# Autodesk Inventor assembly: motor_sima
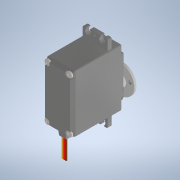
[picture p0: Inventor's stored thumbnail of the model, 180x180]
Saved by Autodesk Inventor 2020.3 (Build 243373000, 373)
## iProperties
Created: 2019-08-01
Part Number: motor_sima
Document SubType Name: Assembly
Designer: Horváth Patrik
Author: Horváth Patrik
## Documents named in this file (3)
- E:\Dokumentumok\Simonyi\INDACT\Robotarm - kézfej fileok\kéz12.0\motor_sima.iam
- E:\Dokumentumok\Simonyi\INDACT\Robotarm - kézfej fileok\kéz12.0\motortarcsa.ipt
- E:\Dokumentumok\Simonyi\INDACT\Robotarm - kézfej fileok\kéz12.0\tower-pro-mg-995-analog-servo-1.snapshot.18\TOWER PRO MG-995, ANALOG SERVO.iam
## Components (2 placed, 2 different names)
1. motortarcsa:1 — Mate:1, Mate:2
2. TOWER PRO MG-995, ANALOG SERVO:1 [sub-assembly] — Mate:1, Mate:2
## Relationships (2: Mate 2)
- Mate:1: motortarcsa:1 ↔ TOWER PRO MG-995, ANALOG SERVO:1
- Mate:2: motortarcsa:1 ↔ TOWER PRO MG-995, ANALOG SERVO:1
